# Autodesk Inventor assembly: halfcut-48t-gear
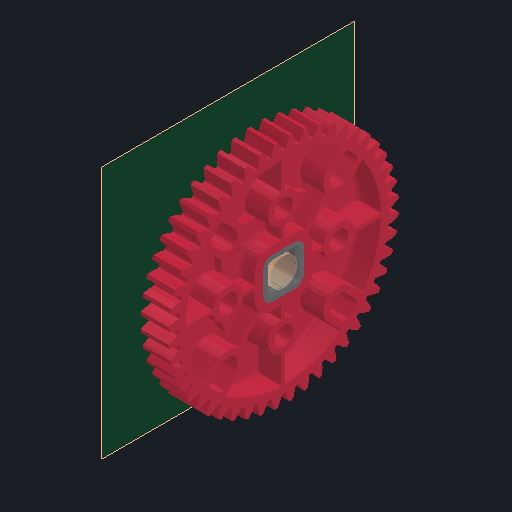
[picture p0: Inventor's stored thumbnail of the model, 512x512]
Saved by Autodesk Inventor 2026.1 (Build 301233000, 233)
## iProperties
Created: 2025-07-20
Part Number: halfcut-48t-gear
Document SubType Name: Assembly
Designer: Exortions
Author: Exortions
## Documents named in this file (3)
- C:\Users\roejo\OneDrive\Documents\2026WorldChampionRobot\Library\VEX-CAD-Inventor-1.4.2\Motion\Gears\HS Gear\halfcut-48t-gear.iam
- C:\Users\roejo\OneDrive\Documents\2026WorldChampionRobot\Library\VEX-CAD-Inventor-1.4.2\Motion\Gears\HS Gear\HS 48T Gear, No Insert.iam
- C:\Users\roejo\OneDrive\Documents\2026WorldChampionRobot\Library\VEX-CAD-Inventor-1.4.2\Motion\Gears\HS Gear.iam
## Components (1 placed, 1 different names)
1. HS 48T Gear, No Insert:1 [sub-assembly] — Flush:1
## Relationships (1: Flush 1)
- Flush:1: HS 48T Gear, No Insert:1
